# Autodesk Inventor assembly: Assembly
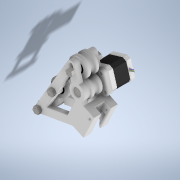
[picture p0: Inventor's stored thumbnail of the model, 180x180]
Saved by Autodesk Inventor 2021 (Build 250183000, 183)
## iProperties
Created: 2021-07-23
Part Number: Assembly
Document SubType Name: Assembly
Designer: zmac845
Author: zmac845
## Documents named in this file (11)
- \\files.auckland.ac.nz\myhome\Documents\Year 4\MECHENG 700\Gao Design Mimic\Inventor Models\10mm Cable\Assembly.iam
- \\files.auckland.ac.nz\myhome\Documents\Year 4\MECHENG 700\Gao Design Mimic\Inventor Models\10mm Cable\DriveWheel_10mm.ipt
- \\files.auckland.ac.nz\myhome\Documents\Year 4\MECHENG 700\Gao Design Mimic\Inventor Models\Nuts & Bolts\M8_Nut.ipt
- \\files.auckland.ac.nz\myhome\Documents\Year 4\MECHENG 700\Gao Design Mimic\Inventor Models\Bearing.ipt
- \\files.auckland.ac.nz\myhome\Documents\Year 4\MECHENG 700\Gao Design Mimic\Inventor Models\M1173041- NEMA 17.ipt
- \\files.auckland.ac.nz\myhome\Documents\Year 4\MECHENG 700\Gao Design Mimic\Inventor Models\10mm Cable\Frame_10mm_stepper.ipt
- \\files.auckland.ac.nz\myhome\Documents\Year 4\MECHENG 700\Gao Design Mimic\Inventor Models\Nuts & Bolts\M3_Bolt_12mm.ipt
- \\files.auckland.ac.nz\myhome\Documents\Year 4\MECHENG 700\Gao Design Mimic\Inventor Models\Nuts & Bolts\M8_Bolt_12mm.ipt
- \\files.auckland.ac.nz\myhome\Documents\Year 4\MECHENG 700\Gao Design Mimic\Inventor Models\Nuts & Bolts\M8_Axle.ipt
- \\files.auckland.ac.nz\myhome\Documents\Year 4\MECHENG 700\Gao Design Mimic\Inventor Models\10mm Cable\AlignWheelHalf_10mm.ipt
- \\files.auckland.ac.nz\myhome\Documents\Year 4\MECHENG 700\Gao Design Mimic\Inventor Models\10mm Cable\LoadedWheel_10mm.ipt
## Components (35 placed, 10 different names)
1. DriveWheel_10mm:1 — Rigid:1
2. M8_Nut:1 — Rigid:1, Rotational:1
3. Bearing:1 — Rotational:1, Rotational:3
4. Frame_10mm_stepper:1 — Rotational:3, Rotational:4, Rotational:8, Rotational:9, Rigid:3, Rotational:10, Rotational:11, Rotational:12, Rotational:13, Rigid:4, Rotational:14, Rotational:15, Rotational:16
5. M1173041- NEMA 17:1 — Rotational:4, Rotational:5, Rotational:6, Rigid:2, Rotational:7
6. M3_Bolt_12mm:1 — Rotational:7
7. M3_Bolt_12mm:2 — Rigid:2
8. M3_Bolt_12mm:3 — Rotational:6
9. M3_Bolt_12mm:4 — Rotational:5
10. M3_Bolt_12mm:5 — Rotational:8
11. M3_Bolt_12mm:6 — Rotational:9
12. M3_Bolt_12mm:7 — Rigid:3
13. M3_Bolt_12mm:8 — Rotational:10
14. M8_Bolt_12mm:1 — Rotational:11
15. M8_Nut:2 — Rotational:16, Rotational:18
16. M8_Nut:3 — Rotational:13
17. M8_Nut:4 — Rotational:12
18. M8_Nut:5 — Rotational:14
19. M8_Nut:6 — Rotational:15, Rotational:19
20. M8_Nut:7 — Rigid:4, Rotational:17
21. M8_Axle:1 — Rotational:19, Cylindrical:2
22. M8_Axle:2 — Rotational:18, Rigid:5, Rigid:6
23. M8_Axle:3 — Rotational:17, Cylindrical:1
24. AlignWheelHalf_10mm:1 — Rigid:6, Rigid:8
25. AlignWheelHalf_10mm:2 — Rigid:5, Rigid:9
26. LoadedWheel_10mm:1 — Cylindrical:1, Rotational:20, Rigid:7
27. Bearing:2 — Rotational:20
28. Bearing:3 — Rigid:7
29. Bearing:4 — Rigid:8
30. Bearing:5 — Rigid:9
31. Bearing:6 — Rotational:23, Rotational:24
32. Bearing:7 — Rotational:21, Rotational:22
33. Bearing:8 — Rotational:22
34. Bearing:9 — Cylindrical:2, Rotational:21, Rotational:23
35. Bearing:10 — Rotational:24
## Relationships (34: RevoluteJoint 23, WeldJoint 9, CylindricalJoint 2)
- Rigid:1 [WeldJoint]: DriveWheel_10mm:1 ↔ M8_Nut:1
- Rotational:1 [RevoluteJoint] (0.5 mm): M8_Nut:1 ↔ Bearing:1
- Rotational:3 [RevoluteJoint] (-0.5 mm): Bearing:1 ↔ Frame_10mm_stepper:1
- Rotational:4 [RevoluteJoint]: Frame_10mm_stepper:1 ↔ M1173041- NEMA 17:1
- Rotational:5 [RevoluteJoint]: M1173041- NEMA 17:1 ↔ M3_Bolt_12mm:4
- Rotational:6 [RevoluteJoint]: M1173041- NEMA 17:1 ↔ M3_Bolt_12mm:3
- Rigid:2 [WeldJoint]: M1173041- NEMA 17:1 ↔ M3_Bolt_12mm:2
- Rotational:7 [RevoluteJoint]: M1173041- NEMA 17:1 ↔ M3_Bolt_12mm:1
- Rotational:8 [RevoluteJoint]: Frame_10mm_stepper:1 ↔ M3_Bolt_12mm:5
- Rotational:9 [RevoluteJoint]: Frame_10mm_stepper:1 ↔ M3_Bolt_12mm:6
- Rigid:3 [WeldJoint]: Frame_10mm_stepper:1 ↔ M3_Bolt_12mm:7
- Rotational:10 [RevoluteJoint]: Frame_10mm_stepper:1 ↔ M3_Bolt_12mm:8
- Rotational:11 [RevoluteJoint]: Frame_10mm_stepper:1 ↔ M8_Bolt_12mm:1
- Rotational:12 [RevoluteJoint]: Frame_10mm_stepper:1 ↔ M8_Nut:4
- Rotational:13 [RevoluteJoint]: Frame_10mm_stepper:1 ↔ M8_Nut:3
- Rigid:4 [WeldJoint] (0.5 mm): Frame_10mm_stepper:1 ↔ M8_Nut:7
- Rotational:14 [RevoluteJoint]: Frame_10mm_stepper:1 ↔ M8_Nut:5
- Rotational:15 [RevoluteJoint]: Frame_10mm_stepper:1 ↔ M8_Nut:6
- Rotational:16 [RevoluteJoint]: Frame_10mm_stepper:1 ↔ M8_Nut:2
- Rotational:17 [RevoluteJoint]: M8_Nut:7 ↔ M8_Axle:3
- Rotational:18 [RevoluteJoint]: M8_Nut:2 ↔ M8_Axle:2
- Rotational:19 [RevoluteJoint]: M8_Nut:6 ↔ M8_Axle:1
- Rigid:5 [WeldJoint]: M8_Axle:2 ↔ AlignWheelHalf_10mm:2
- Rigid:6 [WeldJoint]: M8_Axle:2 ↔ AlignWheelHalf_10mm:1
- Cylindrical:1: M8_Axle:3 ↔ LoadedWheel_10mm:1
- Rotational:20 [RevoluteJoint]: LoadedWheel_10mm:1 ↔ Bearing:2
- Rigid:7 [WeldJoint]: LoadedWheel_10mm:1 ↔ Bearing:3
- Rigid:8 [WeldJoint]: AlignWheelHalf_10mm:1 ↔ Bearing:4
- Rigid:9 [WeldJoint]: AlignWheelHalf_10mm:2 ↔ Bearing:5
- Cylindrical:2: M8_Axle:1 ↔ Bearing:9
- Rotational:21 [RevoluteJoint] (1 mm): Bearing:7 ↔ Bearing:9
- Rotational:22 [RevoluteJoint] (1 mm): Bearing:7 ↔ Bearing:8
- Rotational:23 [RevoluteJoint] (1 mm): Bearing:6 ↔ Bearing:9
- Rotational:24 [RevoluteJoint] (1 mm): Bearing:6 ↔ Bearing:10
